# Autodesk Inventor assembly: IceKeysV1
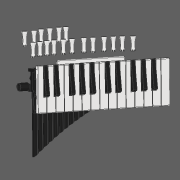
[picture p0: Inventor's stored thumbnail of the model, 180x180]
Saved by Autodesk Inventor 2020 (Build 240168000, 168)
## iProperties
Created: 2019-12-01
Part Number: IceKeysV1
Document SubType Name: Assembly
Designer: Isaac Newcomb
Mass: 617.053 g
Surface Area: 4510.93 cm^2
Volume: 603.079 cm^3
Density: 1.02317 g/cm^3
Project: Ice Keys
Author: Isaac Newcomb
## Documents named in this file (18)
- Z:\Ice Keys\V1\IceKeysV1.iam
- Z:\Ice Keys\V1\Manifold0_Lower.ipt
- Z:\Ice Keys\V1\BlackKey0.ipt
- Z:\Ice Keys\V1\Lever1.ipt
- Z:\Ice Keys\V1\DKey0.ipt
- Z:\Ice Keys\V1\PostValve1_Upper.ipt
- Z:\Ice Keys\V1\PostValve1_Lower.ipt
- Z:\Ice Keys\V1\Manifold0_Upper.ipt
- Z:\Ice Keys\V1\PostValve1.ipt
- Z:\Ice Keys\V1\CKey0.ipt
- Z:\Ice Keys\V1\EKey0.ipt
- Z:\Ice Keys\V1\FKey0.ipt
- Z:\Ice Keys\V1\GKey0.ipt
- Z:\Ice Keys\V1\AKey0.ipt
- Z:\Ice Keys\V1\BKey0.ipt
- Z:\Ice Keys\V1\CKey0_Top.ipt
- Z:\Ice Keys\V1\TuningPlug0.ipt
- Z:\Ice Keys\V1\HandPlate1_Center.ipt
## Components (80 placed, 16 different names)
1. Manifold0_Lower:1 — Rigid:5, Rigid:6, Mate:7, Mate:8, Mate:9
2. PostValve1_Lower:1 — Rigid:4, Rotational:1, Rotational:2, Rigid:5, Mate:4, Mate:5, Mate:6, Rotational:3, Rotational:4, Rotational:5, Rotational:6, Rotational:7, Rotational:9
3. PostValve1_Upper:1 — Rigid:4, Rotational:10, Rotational:8, Cylindrical:2, Cylindrical:3, Cylindrical:4, Cylindrical:5, Cylindrical:6, Cylindrical:9, Cylindrical:7
4. Manifold0_Upper:1 — Rigid:6
5. CKey0_Top:13 — Rotational:8
6. HandPlate1_Center:1 — Mate:7, Mate:8, Mate:9
7. TuningPlug0:1 — Cylindrical:2
8. TuningPlug0:2 — Cylindrical:4
9. TuningPlug0:3 — Cylindrical:3
10. TuningPlug0:4 — Cylindrical:5
11. TuningPlug0:5 — Cylindrical:6
12. TuningPlug0:6 — Cylindrical:9
13. TuningPlug0:7 — Cylindrical:7
14. TuningPlug0:8
15. TuningPlug0:9
16. TuningPlug0:10
17. TuningPlug0:11
18. TuningPlug0:12
19. TuningPlug0:13
20. TuningPlug0:14
21. TuningPlug0:15
22. TuningPlug0:16
23. TuningPlug0:17
24. TuningPlug0:18
25. TuningPlug0:19
26. TuningPlug0:20
27. TuningPlug0:21
28. TuningPlug0:22
29. TuningPlug0:23
30. TuningPlug0:24
31. TuningPlug0:25
32. CKey0:1 — Rotational:3, Rigid:7
33. DKey0:1 — Rotational:2
34. EKey0:2 — Rotational:4
35. FKey0:3 — Rotational:5
36. GKey0:4 — Rotational:6
37. AKey0:5 — Rotational:7
38. BKey0:6 — Rotational:10
39. CKey0:7
40. DKey0:2
41. EKey0:8
42. FKey0:9
43. GKey0:10
44. AKey0:11
45. BKey0:12
46. Lever1:1 — Rigid:7
47. Lever1:2
48. Lever1:3
49. Lever1:4
50. Lever1:5
51. Lever1:6
52. Lever1:7
53. Lever1:8
54. Lever1:9
55. Lever1:10
56. Lever1:11
57. Lever1:12
58. Lever1:13
59. Lever1:14
60. Lever1:15
61. Lever1:16
62. Lever1:17
63. Lever1:18
64. Lever1:19
65. Lever1:20
66. Lever1:21
67. Lever1:22
68. Lever1:23
69. Lever1:24
70. Lever1:25
71. BlackKey0:1 — Rotational:1
72. BlackKey0:2
73. BlackKey0:3 — Rotational:9
74. BlackKey0:4
75. BlackKey0:5
76. BlackKey0:6
77. BlackKey0:7
78. BlackKey0:8
79. BlackKey0:9
80. BlackKey0:10
## Component patterns: White Keys (2 elements), Key Backs (25 elements), Black Keys (2 elements), (2 elements, first: BlackKey0:1), (3 elements, first: BlackKey0:3), Component Pattern 3:2 (2 elements), Component Pattern 4:2 (3 elements)
## Relationships (27: RevoluteJoint 10, CylindricalJoint 7, Mate 6, WeldJoint 4)
- Rigid:4 [WeldJoint]: PostValve1_Lower:1 ↔ PostValve1_Upper:1
- Rotational:1 [RevoluteJoint]: PostValve1_Lower:1 ↔ BlackKey0:1
- Rotational:2 [RevoluteJoint]: PostValve1_Lower:1 ↔ DKey0:1
- Rigid:5 [WeldJoint]: Manifold0_Lower:1 ↔ PostValve1_Lower:1
- Mate:4: PostValve1_Lower:1
- Mate:5: PostValve1_Lower:1
- Mate:6: PostValve1_Lower:1
- Rigid:6 [WeldJoint]: Manifold0_Lower:1 ↔ Manifold0_Upper:1
- Rotational:3 [RevoluteJoint]: PostValve1_Lower:1 ↔ CKey0:1
- Rotational:4 [RevoluteJoint]: PostValve1_Lower:1 ↔ EKey0:2
- Rotational:5 [RevoluteJoint]: PostValve1_Lower:1 ↔ FKey0:3
- Rotational:6 [RevoluteJoint]: PostValve1_Lower:1 ↔ GKey0:4
- Rotational:7 [RevoluteJoint]: PostValve1_Lower:1 ↔ AKey0:5
- Rotational:10 [RevoluteJoint]: PostValve1_Upper:1 ↔ BKey0:6
- Rotational:8 [RevoluteJoint]: PostValve1_Upper:1 ↔ CKey0_Top:13
- Rigid:7 [WeldJoint] (0.1 mm): CKey0:1 ↔ Lever1:1
- Rotational:9 [RevoluteJoint]: PostValve1_Lower:1 ↔ BlackKey0:3
- Cylindrical:2: PostValve1_Upper:1 ↔ TuningPlug0:1
- Mate:7: Manifold0_Lower:1 ↔ HandPlate1_Center:1
- Mate:8: Manifold0_Lower:1 ↔ HandPlate1_Center:1
- Mate:9 (0.3 mm): Manifold0_Lower:1 ↔ HandPlate1_Center:1
- Cylindrical:3: PostValve1_Upper:1 ↔ TuningPlug0:3
- Cylindrical:4: PostValve1_Upper:1 ↔ TuningPlug0:2
- Cylindrical:5: PostValve1_Upper:1 ↔ TuningPlug0:4
- Cylindrical:6: PostValve1_Upper:1 ↔ TuningPlug0:5
- Cylindrical:9: PostValve1_Upper:1 ↔ TuningPlug0:6
- Cylindrical:7: PostValve1_Upper:1 ↔ TuningPlug0:7
## Named parameters: chanWidth = 12 mm, keyCount = 25, resoWallThick = 0.75 mm
